# Autodesk Inventor assembly: LandingGearNose2
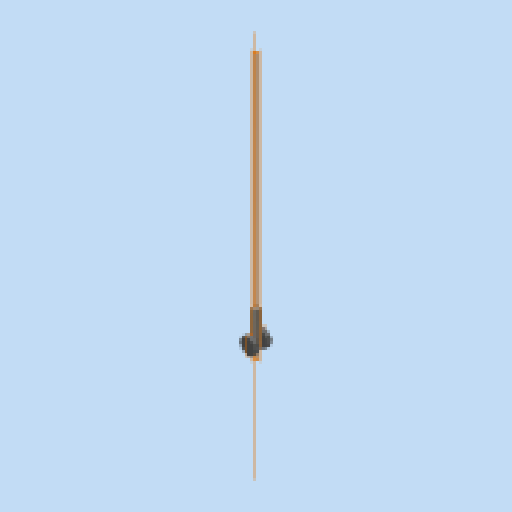
[picture p0: Inventor's stored thumbnail of the model, 512x512]
Saved by Autodesk Inventor 2026.1 (Build 301233000, 233)
## iProperties
Created: 2026-03-19
Part Number: LandingGearNose2
Document SubType Name: Assembly
Designer: mateo
Author: mateo
## Documents named in this file (3)
- C:\GitHub\Senior-Design-UAV\Elytra CAD\Parts\Landing Gear\V2\LandingGearNose2.iam
- C:\GitHub\Senior-Design-UAV\Elytra CAD\Parts\Landing Gear\V2\20x20x130ExtrudedAluminum.ipt
- C:\GitHub\Senior-Design-UAV\Elytra CAD\Parts\Landing Gear\V2\wheel.ipt
## Components (3 placed, 2 different names)
1. 20x20x130ExtrudedAluminum:1 — Mate:1, Mate:2, Mate:3, Mate:4
2. wheel:1 — Mate:3, Mate:4
3. wheel:2 — Mate:1, Mate:2
## Relationships (4: Mate 4)
- Mate:1: 20x20x130ExtrudedAluminum:1 ↔ wheel:2
- Mate:2 (2 mm): 20x20x130ExtrudedAluminum:1 ↔ wheel:2
- Mate:3: 20x20x130ExtrudedAluminum:1 ↔ wheel:1
- Mate:4 (2 mm): 20x20x130ExtrudedAluminum:1 ↔ wheel:1
